# Autodesk Inventor assembly: Display Assembly
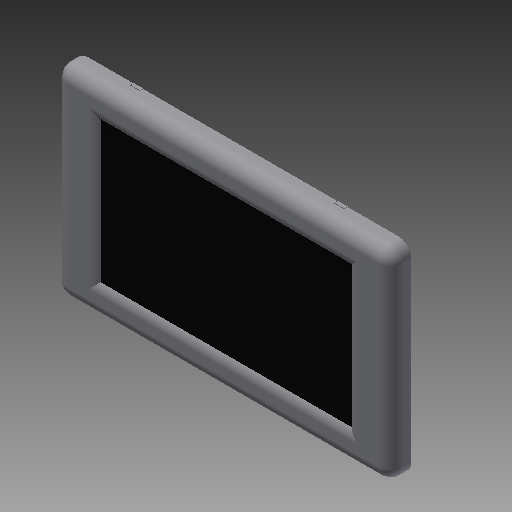
[picture p0: Inventor's stored thumbnail of the model, 512x512]
Saved by Autodesk Inventor 2018 (Build 220112000, 112)
## iProperties
Created: 2019-11-11
Part Number: Display Assembly
Document SubType Name: Assembly
Designer: Jacob
Author: Jacob
## Documents named in this file (7)
- C:\Users\Jacob\git_repos\POE-AIO\CAD Files\New Parts\Display Assembly.iam
- C:\Users\Jacob\git_repos\POE-AIO\CAD Files\Official parts\raspberry pi display.ipt
- C:\Users\Jacob\git_repos\POE-AIO\CAD Files\Better designed front piece.ipt
- C:\Users\Jacob\git_repos\POE-AIO\CAD Files\better support stick.ipt
- C:\Users\Jacob\git_repos\POE-AIO\CAD Files\Official parts\Raspberry Pi 3 .ipt
- C:\Users\Jacob\git_repos\POE-AIO\CAD Files\Official parts\Stand off.ipt
- C:\Users\Jacob\git_repos\POE-AIO\CAD Files\Official parts\raspberry pi display module.ipt
## Components (10 placed, 6 different names)
1. raspberry pi display:1
2. Better designed front piece:1
3. better support stick:1
4. better support stick:2
5. Raspberry Pi 3 :1
6. Stand off:1
7. Stand off:2
8. Stand off:3
9. Stand off:4
10. raspberry pi display module:1
## Relationships (23: Mate 23)
- [Mate] (1 mm): raspberry pi display:1 ↔ Better designed front piece:1
- [Mate]: raspberry pi display:1 ↔ Better designed front piece:1
- [Mate] (0.5 mm): raspberry pi display:1 ↔ Better designed front piece:1
- [Mate]: raspberry pi display:1 ↔ better support stick:1
- [Mate]: raspberry pi display:1 ↔ better support stick:1
- [Mate]: raspberry pi display:1 ↔ better support stick:2
- [Mate]: raspberry pi display:1 ↔ better support stick:2
- [Mate]: raspberry pi display:1 ↔ better support stick:1
- [Mate]: raspberry pi display:1 ↔ raspberry pi display module:1
- [Mate]: raspberry pi display:1 ↔ raspberry pi display module:1
- [Mate]: raspberry pi display:1 ↔ raspberry pi display module:1
- [Mate]: Stand off:2 ↔ raspberry pi display module:1
- [Mate]: Stand off:2 ↔ raspberry pi display module:1
- [Mate]: Stand off:1 ↔ raspberry pi display module:1
- [Mate]: Stand off:1 ↔ raspberry pi display module:1
- [Mate]: Stand off:3 ↔ raspberry pi display module:1
- [Mate]: Stand off:3 ↔ raspberry pi display module:1
- [Mate]: Stand off:4 ↔ raspberry pi display module:1
- [Mate]: Stand off:4 ↔ raspberry pi display module:1
- [Mate]: Raspberry Pi 3 :1 ↔ Stand off:2
- [Mate]: Raspberry Pi 3 :1 ↔ Stand off:1
- [Mate]: Raspberry Pi 3 :1 ↔ Stand off:4
- [Mate]: raspberry pi display:1 ↔ better support stick:2
